# Autodesk Inventor assembly: Assembly146-01
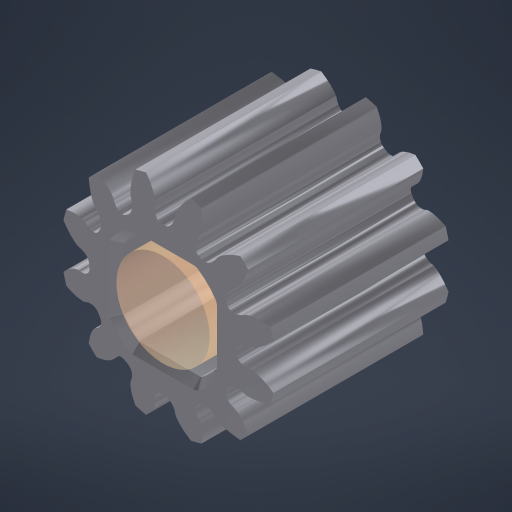
[picture p0: Inventor's stored thumbnail of the model, 512x512]
Saved by Autodesk Inventor 2023.2 (Build 272271000, 271)
## iProperties
Created: 2022-08-02
Part Number: Assembly146-01
Document SubType Name: Assembly
Designer: ylu12
Author: ylu12
## Documents named in this file (3)
- D:\CAD\Parts\standard\Motion\Gears\HS\HS 12T Gear, No Insert.iam
- D:\CAD\Parts\standard\Motion\Gears\HS\Reference parts\HS 12T Gear, No Insert.ipt
- D:\CAD\Parts\standard\Motion\Gears\HS\HS Gear.iam
## Components (1 placed, 1 different names)
1. 12T — Mate:5, Mate:6, Flush:3
## Relationships (3: Mate 2, Flush 1)
- Mate:5: 12T
- Mate:6: 12T
- Flush:3: 12T
